# Autodesk Inventor assembly: Assembly1
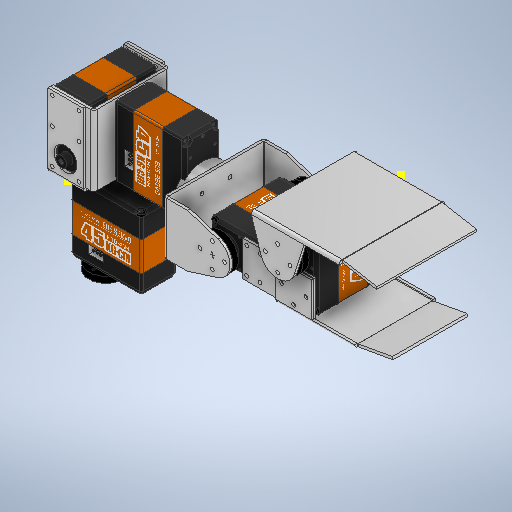
[picture p0: Inventor's stored thumbnail of the model, 512x512]
Saved by Autodesk Inventor 2025.2 (Build 292293000, 293)
## iProperties
Created: 2025-05-12
Part Number: Assembly1
Document SubType Name: Assembly
Designer: LG
Author: LG
## Documents named in this file (12)
- C:\Users\LG\Desktop\RHp_Humanoid_ver1\Assembly\6_right_Arm.iam
- C:\Users\LG\Desktop\RHp_Humanoid_ver1\Part\HTD-45H, Horn\HTD-45H Assembly.iam
- C:\Users\LG\Desktop\RHp_Humanoid_ver1\Part\Frame\Arm\axis_19_top_frame.ipt
- C:\Users\LG\Desktop\RHp_Humanoid_ver1\Part\HTD-45H, Horn\HTD-45H\HTD-45H.ipt
- C:\Users\LG\Desktop\RHp_Humanoid_ver1\Part\Frame\Arm\axis_20_bottom_frame.ipt
- C:\Users\LG\Desktop\RHp_Humanoid_ver1\Part\HTD-45H, Horn\Horn\Top Horn.ipt
- C:\Users\LG\Desktop\RHp_Humanoid_ver1\Part\Frame\Arm\axis_4_top_frame.ipt
- C:\Users\LG\Desktop\RHp_Humanoid_ver1\Part\Frame\Arm\axis_21_bottom_frame.ipt
- C:\Users\LG\Desktop\RHp_Humanoid_ver1\Part\Frame\Arm\axis_22_top_frame(middle).ipt
- C:\Users\LG\Desktop\RHp_Humanoid_ver1\Part\Frame\Arm\axis_22_bottom_frame(middle).ipt
- C:\Users\LG\Desktop\RHp_Humanoid_ver1\Part\Frame\Arm\axis_24_bottom_frame.ipt
- C:\Users\LG\Desktop\RHp_Humanoid_ver1\Part\Frame\Arm\axis_24_top_frame.ipt
## Components (14 placed, 11 different names)
1. HTD-45H Assembly:1 [sub-assembly] — Mate:26, Flush:12, Mate:27, Flush:15, Flush:16, Flush:17
2. axis_19_top_frame:1 — Mate:26, Flush:12, Mate:27, Flush:13, Flush:14, Mate:28
3. HTD-45H:1 — Mate:4, Mate:6, Mate:7, Flush:13, Flush:14, Mate:28, Mate:29
4. axis_20_bottom_frame:1 — Mate:4, Mate:6, Mate:7, Mate:10, Mate:11, Mate:12, Mate:29
5. HTD-45H:2 — Mate:10, Mate:11, Mate:12, Mate:13, Mate:14, Flush:4, Mate:15, Mate:17
6. axis_4_top_frame:1 — Mate:13, Mate:14, Flush:4, Mate:16, Flush:18, Mate:30, Flush:19
7. Top Horn:1 — Mate:15, Mate:16, Mate:17
8. axis_21_bottom_frame:1 — Mate:20, Mate:21, Mate:22, Flush:18, Mate:30, Flush:19
9. HTD-45H Assembly:2 [sub-assembly] — Mate:20, Mate:21, Mate:22, Flush:9, Mate:31, Flush:20, Flush:21
10. axis_22_top_frame(middle):1 — Flush:9, Flush:22, Flush:23, Mate:32
11. axis_22_bottom_frame(middle):1 — Flush:24, Flush:25, Mate:33, Mate:37, Flush:27
12. HTD-45H Assembly:3 [sub-assembly] — Mate:31, Flush:20, Flush:21, Flush:22, Flush:23, Mate:32, Flush:24, Flush:25, Mate:33, Mate:34, Mate:35, Flush:26, Mate:36
13. axis_24_bottom_frame:1 — Mate:34, Mate:35, Flush:26
14. axis_24_top_frame:1 — Mate:36, Mate:37, Flush:27
## Relationships (44: Mate 26, Flush 18)
- Mate:4: HTD-45H:1 ↔ axis_20_bottom_frame:1
- Mate:6: HTD-45H:1 ↔ axis_20_bottom_frame:1
- Mate:7: HTD-45H:1 ↔ axis_20_bottom_frame:1
- Mate:10: axis_20_bottom_frame:1 ↔ HTD-45H:2
- Mate:11: axis_20_bottom_frame:1 ↔ HTD-45H:2
- Mate:12: axis_20_bottom_frame:1 ↔ HTD-45H:2
- Mate:13: HTD-45H:2 ↔ axis_4_top_frame:1
- Mate:14: HTD-45H:2 ↔ axis_4_top_frame:1
- Flush:4: HTD-45H:2 ↔ axis_4_top_frame:1
- Mate:15: HTD-45H:2 ↔ Top Horn:1
- Mate:16: axis_4_top_frame:1 ↔ Top Horn:1
- Mate:17: HTD-45H:2 ↔ Top Horn:1
- Mate:20: axis_21_bottom_frame:1 ↔ HTD-45H Assembly:2
- Mate:21 (16.43 mm): axis_21_bottom_frame:1 ↔ HTD-45H Assembly:2
- Mate:22: axis_21_bottom_frame:1 ↔ HTD-45H Assembly:2
- Flush:9: HTD-45H Assembly:2 ↔ axis_22_top_frame(middle):1
- Mate:26: HTD-45H Assembly:1 ↔ axis_19_top_frame:1
- Flush:12: HTD-45H Assembly:1 ↔ axis_19_top_frame:1
- Mate:27: HTD-45H Assembly:1 ↔ axis_19_top_frame:1
- Flush:13: axis_19_top_frame:1 ↔ HTD-45H:1
- Flush:14: axis_19_top_frame:1 ↔ HTD-45H:1
- Mate:28: axis_19_top_frame:1 ↔ HTD-45H:1
- Flush:15: HTD-45H Assembly:1
- Flush:16: HTD-45H Assembly:1
- Flush:17: HTD-45H Assembly:1
- Mate:29 (3 mm): HTD-45H:1 ↔ axis_20_bottom_frame:1
- Flush:18: axis_4_top_frame:1 ↔ axis_21_bottom_frame:1
- Mate:30: axis_4_top_frame:1 ↔ axis_21_bottom_frame:1
- Flush:19: axis_4_top_frame:1 ↔ axis_21_bottom_frame:1
- Mate:31: HTD-45H Assembly:2 ↔ HTD-45H Assembly:3
- Flush:20: HTD-45H Assembly:2 ↔ HTD-45H Assembly:3
- Flush:21: HTD-45H Assembly:2 ↔ HTD-45H Assembly:3
- Flush:22: axis_22_top_frame(middle):1 ↔ HTD-45H Assembly:3
- Flush:23: axis_22_top_frame(middle):1 ↔ HTD-45H Assembly:3
- Mate:32: axis_22_top_frame(middle):1 ↔ HTD-45H Assembly:3
- Flush:24: axis_22_bottom_frame(middle):1 ↔ HTD-45H Assembly:3
- Flush:25: axis_22_bottom_frame(middle):1 ↔ HTD-45H Assembly:3
- Mate:33: axis_22_bottom_frame(middle):1 ↔ HTD-45H Assembly:3
- Mate:34: HTD-45H Assembly:3 ↔ axis_24_bottom_frame:1
- Mate:35 (4.43 mm): HTD-45H Assembly:3 ↔ axis_24_bottom_frame:1
- Flush:26 (-10 mm): HTD-45H Assembly:3 ↔ axis_24_bottom_frame:1
- Mate:36: HTD-45H Assembly:3 ↔ axis_24_top_frame:1
- Mate:37: axis_22_bottom_frame(middle):1 ↔ axis_24_top_frame:1
- Flush:27: axis_22_bottom_frame(middle):1 ↔ axis_24_top_frame:1
